# Autodesk Inventor assembly: Cylinder
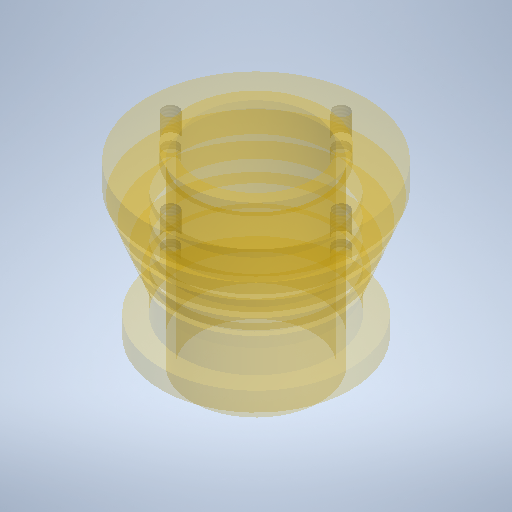
[picture p0: Inventor's stored thumbnail of the model, 512x512]
Saved by Autodesk Inventor 2025 (Build 290162010, 162A)
## iProperties
Created: 2024-07-17
Part Number: Cylinder
Document SubType Name: Assembly
Designer: ffogue
Author: ffogue
## Documents named in this file (3)
- C:\Users\ffogue\OneDrive - MuM - OM\Dokumente\Inventor\Boxermotor\Cylinder.iam
- C:\Users\ffogue\OneDrive - MuM - OM\Dokumente\Inventor\Boxermotor\gehaeuse.ipt
- C:\Users\ffogue\OneDrive - MuM - OM\Dokumente\Inventor\Boxermotor\gehaeuse2.ipt
## Components (2 placed, 2 different names)
1. gehaeuse:1 — Mate:1, Insert:1
2. gehaeuse2:1 — Mate:1, Insert:1
## Relationships (2: Mate 1, Insert 1)
- Mate:1: gehaeuse:1 ↔ gehaeuse2:1
- Insert:1: gehaeuse:1 ↔ gehaeuse2:1
